# Autodesk Inventor assembly: chain(a)
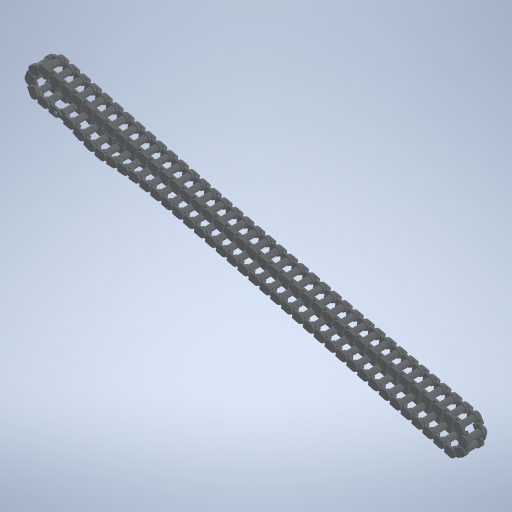
[picture p0: Inventor's stored thumbnail of the model, 512x512]
Saved by Autodesk Inventor 2023 (Build 270158000, 158)
## iProperties
Created: 2022-08-08
Part Number: chain(a)
Document SubType Name: Assembly
Designer: aaron
Author: aaron
## Documents named in this file (3)
- C:\Users\aaron\Documents\Inventor\Spin Up\library\Motion\New Sprockets\chain(a2).iam
- C:\Users\aaron\Documents\Inventor\Spin Up\library\Motion\New Sprockets\IQ chain.ipt
- C:\Users\aaron\Documents\Inventor\Spin Up\library\Motion\New Sprockets\8T.ipt
## Components (84 placed, 2 different names)
1. IQ chain:1 — Mate:2, Flush:3, Mate:64, Flush:65
2. IQ chain:2 — Mate:2, Flush:3, Mate:4, Flush:5
3. IQ chain:3 — Mate:4, Flush:5
4. IQ chain:4 — Mate:8, Flush:9
5. IQ chain:5 — Mate:8, Flush:9
6. IQ chain:6
7. IQ chain:7
8. IQ chain:8 — Mate:16, Flush:17
9. IQ chain:9 — Mate:16, Flush:17
10. IQ chain:10
11. IQ chain:11
12. IQ chain:12
13. IQ chain:13
14. IQ chain:14
15. IQ chain:15
16. IQ chain:16 — Mate:32, Flush:33
17. IQ chain:17 — Mate:32, Flush:33
18. IQ chain:18
19. IQ chain:19
20. IQ chain:20
21. IQ chain:21
22. IQ chain:22
23. IQ chain:23
24. IQ chain:24
25. IQ chain:25 — Mate:113, Flush:94
26. IQ chain:27 — Mate:113
27. IQ chain:28 — Flush:94
28. IQ chain:29 — Mate:120, Mate:125
29. IQ chain:33 — Mate:100, Flush:84
30. IQ chain:34
31. IQ chain:35
32. IQ chain:36
33. IQ chain:37
34. IQ chain:38
35. IQ chain:39
36. IQ chain:40
37. IQ chain:41
38. IQ chain:42
39. IQ chain:43
40. IQ chain:44
41. IQ chain:45
42. IQ chain:46
43. IQ chain:47
44. IQ chain:48
45. IQ chain:49
46. IQ chain:50
47. IQ chain:51 — Mate:118
48. IQ chain:52 — Mate:115
49. IQ chain:53 — Mate:116
50. IQ chain:54 — Mate:117
51. IQ chain:55
52. IQ chain:56
53. IQ chain:57
54. IQ chain:58
55. IQ chain:59
56. IQ chain:60
57. IQ chain:61
58. IQ chain:62
59. IQ chain:63
60. IQ chain:64 — Mate:64, Flush:65
61. IQ chain:70 — Mate:124, Mate:125
62. IQ chain:71 — Mate:122
63. IQ chain:72 — Mate:123
64. IQ chain:73 — Flush:95, Tangent:1
65. IQ chain:75 — Flush:95, Tangent:1
66. IQ chain:76 — Mate:109, Flush:93
67. IQ chain:77 — Mate:108, Flush:92
68. IQ chain:78
69. IQ chain:79
70. IQ chain:80
71. IQ chain:81
72. IQ chain:82
73. IQ chain:83 — Mate:100, Flush:84
74. IQ chain:84 — Mate:108, Flush:92
75. IQ chain:85 — Mate:110
76. IQ chain:86
77. IQ chain:87
78. IQ chain:88
79. IQ chain:89
80. IQ chain:90
81. IQ chain:91
82. IQ chain:92 — Mate:109, Flush:93, Mate:110
83. 8T:1 — Mate:114, Mate:115, Mate:116, Mate:117, Mate:118
84. 8T:2 — Mate:114, Mate:120, Mate:122, Mate:123, Mate:124
## Relationships (171: Mate 90, Flush 80, Tangent 1)
- Mate:2: IQ chain:1 ↔ IQ chain:2
- Flush:3: IQ chain:1 ↔ IQ chain:2
- [Mate]: IQ chain:3 ↔ IQ chain:4
- [Flush]: IQ chain:3 ↔ IQ chain:4
- Mate:4: IQ chain:2 ↔ IQ chain:3
- Flush:5: IQ chain:2 ↔ IQ chain:3
- [Mate]: IQ chain:5 ↔ IQ chain:6
- [Flush]: IQ chain:5 ↔ IQ chain:6
- [Mate]: IQ chain:7 ↔ IQ chain:8
- [Flush]: IQ chain:7 ↔ IQ chain:8
- [Mate]: IQ chain:6 ↔ IQ chain:7
- [Flush]: IQ chain:6 ↔ IQ chain:7
- Mate:8: IQ chain:4 ↔ IQ chain:5
- Flush:9: IQ chain:4 ↔ IQ chain:5
- [Mate]: IQ chain:9 ↔ IQ chain:10
- [Flush]: IQ chain:9 ↔ IQ chain:10
- [Mate]: IQ chain:11 ↔ IQ chain:12
- [Flush]: IQ chain:11 ↔ IQ chain:12
- [Mate]: IQ chain:10 ↔ IQ chain:11
- [Flush]: IQ chain:10 ↔ IQ chain:11
- [Mate]: IQ chain:13 ↔ IQ chain:14
- [Flush]: IQ chain:13 ↔ IQ chain:14
- [Mate]: IQ chain:15 ↔ IQ chain:16
- [Flush]: IQ chain:15 ↔ IQ chain:16
- [Mate]: IQ chain:14 ↔ IQ chain:15
- [Flush]: IQ chain:14 ↔ IQ chain:15
- [Mate]: IQ chain:12 ↔ IQ chain:13
- [Flush]: IQ chain:12 ↔ IQ chain:13
- Mate:16: IQ chain:8 ↔ IQ chain:9
- Flush:17: IQ chain:8 ↔ IQ chain:9
- [Mate]: IQ chain:17 ↔ IQ chain:18
- [Flush]: IQ chain:17 ↔ IQ chain:18
- [Mate]: IQ chain:19 ↔ IQ chain:20
- [Flush]: IQ chain:19 ↔ IQ chain:20
- [Mate]: IQ chain:18 ↔ IQ chain:19
- [Flush]: IQ chain:18 ↔ IQ chain:19
- [Mate]: IQ chain:21 ↔ IQ chain:22
- [Flush]: IQ chain:21 ↔ IQ chain:22
- [Mate]: IQ chain:23 ↔ IQ chain:24
- [Flush]: IQ chain:23 ↔ IQ chain:24
- [Mate]: IQ chain:22 ↔ IQ chain:23
- [Flush]: IQ chain:22 ↔ IQ chain:23
- [Mate]: IQ chain:20 ↔ IQ chain:21
- [Flush]: IQ chain:20 ↔ IQ chain:21
- [Mate]: IQ chain:27 ↔ IQ chain:28
- [Flush]: IQ chain:27 ↔ IQ chain:28
- [Mate]: IQ chain:28 ↔ IQ chain:29
- [Flush]: IQ chain:28 ↔ IQ chain:29
- [Mate]: IQ chain:24 ↔ IQ chain:25
- [Flush]: IQ chain:24 ↔ IQ chain:25
- Mate:32: IQ chain:16 ↔ IQ chain:17
- Flush:33: IQ chain:16 ↔ IQ chain:17
- [Mate]: IQ chain:33 ↔ IQ chain:34
- [Flush]: IQ chain:33 ↔ IQ chain:34
- [Mate]: IQ chain:35 ↔ IQ chain:36
- [Flush]: IQ chain:35 ↔ IQ chain:36
- [Mate]: IQ chain:34 ↔ IQ chain:35
- [Flush]: IQ chain:34 ↔ IQ chain:35
- [Mate]: IQ chain:37 ↔ IQ chain:38
- [Flush]: IQ chain:37 ↔ IQ chain:38
- [Mate]: IQ chain:39 ↔ IQ chain:40
- [Flush]: IQ chain:39 ↔ IQ chain:40
- [Mate]: IQ chain:38 ↔ IQ chain:39
- [Flush]: IQ chain:38 ↔ IQ chain:39
- [Mate]: IQ chain:36 ↔ IQ chain:37
- [Flush]: IQ chain:36 ↔ IQ chain:37
- [Mate]: IQ chain:41 ↔ IQ chain:42
- [Flush]: IQ chain:41 ↔ IQ chain:42
- [Mate]: IQ chain:43 ↔ IQ chain:44
- [Flush]: IQ chain:43 ↔ IQ chain:44
- [Mate]: IQ chain:42 ↔ IQ chain:43
- [Flush]: IQ chain:42 ↔ IQ chain:43
- [Mate]: IQ chain:45 ↔ IQ chain:46
- [Flush]: IQ chain:45 ↔ IQ chain:46
- [Mate]: IQ chain:47 ↔ IQ chain:48
- [Flush]: IQ chain:47 ↔ IQ chain:48
- [Mate]: IQ chain:46 ↔ IQ chain:47
- [Flush]: IQ chain:46 ↔ IQ chain:47
- [Mate]: IQ chain:44 ↔ IQ chain:45
- [Flush]: IQ chain:44 ↔ IQ chain:45
- [Mate]: IQ chain:40 ↔ IQ chain:41
- [Flush]: IQ chain:40 ↔ IQ chain:41
- [Mate]: IQ chain:49 ↔ IQ chain:50
- [Flush]: IQ chain:49 ↔ IQ chain:50
- [Mate]: IQ chain:51 ↔ IQ chain:52
- [Flush]: IQ chain:51 ↔ IQ chain:52
- [Mate]: IQ chain:50 ↔ IQ chain:51
- [Flush]: IQ chain:50 ↔ IQ chain:51
- [Mate]: IQ chain:53 ↔ IQ chain:54
- [Flush]: IQ chain:53 ↔ IQ chain:54
- [Mate]: IQ chain:55 ↔ IQ chain:56
- [Flush]: IQ chain:55 ↔ IQ chain:56
- [Mate]: IQ chain:54 ↔ IQ chain:55
- [Flush]: IQ chain:54 ↔ IQ chain:55
- [Mate]: IQ chain:52 ↔ IQ chain:53
- [Flush]: IQ chain:52 ↔ IQ chain:53
- [Mate]: IQ chain:57 ↔ IQ chain:58
- [Flush]: IQ chain:57 ↔ IQ chain:58
- [Mate]: IQ chain:59 ↔ IQ chain:60
- [Flush]: IQ chain:59 ↔ IQ chain:60
- [Mate]: IQ chain:58 ↔ IQ chain:59
- [Flush]: IQ chain:58 ↔ IQ chain:59
- [Mate]: IQ chain:61 ↔ IQ chain:62
- [Flush]: IQ chain:61 ↔ IQ chain:62
- [Mate]: IQ chain:63 ↔ IQ chain:64
- [Flush]: IQ chain:63 ↔ IQ chain:64
- [Mate]: IQ chain:62 ↔ IQ chain:63
- [Flush]: IQ chain:62 ↔ IQ chain:63
- [Mate]: IQ chain:60 ↔ IQ chain:61
- [Flush]: IQ chain:60 ↔ IQ chain:61
- [Mate]: IQ chain:56 ↔ IQ chain:57
- [Flush]: IQ chain:56 ↔ IQ chain:57
- [Mate]: IQ chain:48 ↔ IQ chain:49
- [Flush]: IQ chain:48 ↔ IQ chain:49
- Mate:64: IQ chain:1 ↔ IQ chain:64
- Flush:65: IQ chain:1 ↔ IQ chain:64
- [Mate]: IQ chain:70 ↔ IQ chain:71
- [Flush]: IQ chain:70 ↔ IQ chain:71
- [Mate]: IQ chain:72 ↔ IQ chain:73
- [Flush]: IQ chain:72 ↔ IQ chain:73
- [Mate]: IQ chain:71 ↔ IQ chain:72
- [Flush]: IQ chain:71 ↔ IQ chain:72
- [Mate]: IQ chain:75 ↔ IQ chain:76
- [Flush]: IQ chain:75 ↔ IQ chain:76
- [Mate]: IQ chain:77 ↔ IQ chain:78
- [Flush]: IQ chain:77 ↔ IQ chain:78
- [Mate]: IQ chain:79 ↔ IQ chain:80
- [Flush]: IQ chain:79 ↔ IQ chain:80
- [Mate]: IQ chain:78 ↔ IQ chain:79
- [Flush]: IQ chain:78 ↔ IQ chain:79
- [Mate]: IQ chain:81 ↔ IQ chain:82
- [Flush]: IQ chain:81 ↔ IQ chain:82
- [Mate]: IQ chain:82 ↔ IQ chain:83
- [Flush]: IQ chain:82 ↔ IQ chain:83
- [Mate]: IQ chain:80 ↔ IQ chain:81
- [Flush]: IQ chain:80 ↔ IQ chain:81
- Mate:100: IQ chain:33 ↔ IQ chain:83
- Flush:84: IQ chain:33 ↔ IQ chain:83
- [Mate]: IQ chain:85 ↔ IQ chain:86
- [Flush]: IQ chain:85 ↔ IQ chain:86
- [Mate]: IQ chain:87 ↔ IQ chain:88
- [Flush]: IQ chain:87 ↔ IQ chain:88
- [Mate]: IQ chain:86 ↔ IQ chain:87
- [Flush]: IQ chain:86 ↔ IQ chain:87
- [Mate]: IQ chain:89 ↔ IQ chain:90
- [Flush]: IQ chain:89 ↔ IQ chain:90
- [Mate]: IQ chain:90 ↔ IQ chain:91
- [Flush]: IQ chain:90 ↔ IQ chain:91
- [Mate]: IQ chain:88 ↔ IQ chain:89
- [Flush]: IQ chain:88 ↔ IQ chain:89
- [Mate]: IQ chain:84 ↔ IQ chain:91
- [Flush]: IQ chain:84 ↔ IQ chain:91
- Mate:108: IQ chain:77 ↔ IQ chain:84
- Flush:92: IQ chain:77 ↔ IQ chain:84
- Mate:109: IQ chain:76 ↔ IQ chain:92
- Flush:93: IQ chain:76 ↔ IQ chain:92
- Mate:110: IQ chain:85 ↔ IQ chain:92
- Mate:113: IQ chain:25 ↔ IQ chain:27
- Mate:114 (235.712 mm): 8T:1 ↔ 8T:2
- Mate:115: IQ chain:52 ↔ 8T:1
- Mate:116: IQ chain:53 ↔ 8T:1
- Mate:117: IQ chain:54 ↔ 8T:1
- Mate:118: IQ chain:51 ↔ 8T:1
- Flush:94: IQ chain:25 ↔ IQ chain:28
- Mate:120: IQ chain:29 ↔ 8T:2
- Mate:122: IQ chain:71 ↔ 8T:2
- Mate:123: IQ chain:72 ↔ 8T:2
- Mate:124: IQ chain:70 ↔ 8T:2
- Mate:125: IQ chain:29 ↔ IQ chain:70
- Flush:95: IQ chain:73 ↔ IQ chain:75
- Tangent:1: IQ chain:73 ↔ IQ chain:75
## Named parameters: d5_d3 = 0 mm, d6_d4 = 0 mm, d9_d3 = 0 mm, d10_d4 = 0 mm, d11_d5_d3 = 0 mm, d12_d6_d4 = 0 mm, d13_d7 = 0 mm, d14_d8 = 0 mm, d17_d3 = 0 mm, d18_d4 = 0 mm, d19_d5_d3 = 0 mm, d20_d6_d4 = 0 mm, d21_d7 = 0 mm, d22_d8 = 0 mm, d23_d9_d3 = 0 mm, d24_d10_d4 = 0 mm, d25_d11_d5_d3 = 0 mm, d26_d12_d6_d4 = 0 mm, d27_d13_d7 = 0 mm, d28_d14_d8 = 0 mm, d29_d15 = 0 mm, d30_d16 = 0 mm, d33_d32 = 0 mm, d34_d3 = 0 mm, d35_d4 = 0 mm, d36_d5_d3 = 0 mm, d37_d6_d4 = 0 mm, d38_d7 = 0 mm, d39_d8 = 0 mm, d40_d9_d3 = 0 mm, d41_d10_d4 = 0 mm, d42_d11_d5_d3 = 0 mm, d43_d12_d6_d4 = 0 mm, d44_d13_d7 = 0 mm, d45_d14_d8 = 0 mm, d46_d15 = 0 mm, d47_d16 = 0 mm, d50_d19_d5_d3 = 0 mm, d51_d20_d6_d4 = 0 mm, d60_d29_d15 = 0 mm, d61_d30_d16 = 0 mm, d62_d31 = 0 mm, d65_d32 = 0 mm, d66_d33_d32 = 0 mm, d67_d34_d3 = 0 mm, d68_d35_d4 = 0 mm, d69_d36_d5_d3 = 0 mm, d70_d37_d6_d4 = 0 mm, d71_d38_d7 = 0 mm, d72_d39_d8 = 0 mm, d73_d40_d9_d3 = 0 mm, d74_d41_d10_d4 = 0 mm, d75_d42_d11_d5_d3 = 0 mm, d76_d43_d12_d6_d4 = 0 mm, d77_d44_d13_d7 = 0 mm, d78_d45_d14_d8 = 0 mm, d79_d46_d15 = 0 mm, d80_d47_d16 = 0 mm, d81_d48_d17_d3 = 0 mm, d82_d49_d18_d4 = 0 mm, d83_d50_d19_d5_d3 = 0 mm, d84_d51_d20_d6_d4 = 0 mm, d85_d52_d21_d7 = 0 mm, d86_d53_d22_d8 = 0 mm, d87_d54_d23_d9_d3 = 0 mm, d88_d55_d24_d10_d4 = 0 mm, d89_d56_d25_d11_d5_d3 = 0 mm, d90_d57_d26_d12_d6_d4 = 0 mm, d91_d58_d27_d13_d7 = 0 mm, d92_d59_d28_d14_d8 = 0 mm, d93_d60_d29_d15 = 0 mm, d94_d61_d30_d16 = 0 mm, d95_d62_d31 = 0 mm, d96_d63 = 0 mm, d97_d64 = 0 mm, d98_d3 = 0 mm, d99_d4 = 0 mm, d100_d5_d3 = 0 mm, d101_d6_d4 = 0 mm, d102_d7 = 0 mm, d103_d8 = 0 mm, d104_d9_d3 = 0 mm, d105_d10_d4 = 0 mm, d106_d11_d5_d3 = 0 mm, d107_d12_d6_d4 = 0 mm, d108_d13_d7 = 0 mm, d109_d14_d8 = 0 mm, d110_d15 = 0 mm, d111_d16 = 0 mm, d112_d17_d3 = 0 mm, d113_d18_d4 = 0 mm, d114_d19_d5_d3 = 0 mm, d115_d20_d6_d4 = 0 mm, d116_d21_d7 = 0 mm, d117_d22_d8 = 0 mm, d118_d23_d9_d3 = 0 mm, d119_d24_d10_d4 = 0 mm, d120_d25_d11_d5_d3 = 0 mm, d121_d26_d12_d6_d4 = 0 mm, d122_d27_d13_d7 = 0 mm, d123_d28_d14_d8 = 0 mm, d124_d29_d15 = 0 mm, d125_d30_d16 = 0 mm, d126_d31 = 0 mm, d136_d38_d7 = 0 mm, d137_d39_d8 = 0 mm, d146_d23_d9_d3 = 0 mm, d147_d24_d10_d4 = 0 mm, d148_d25_d11_d5_d3 = 0 mm, d149_d26_d12_d6_d4 = 0 mm, d150_d27_d13_d7 = 0 mm, d151_d28_d14_d8 = 0 mm, d170_d98_d3 = 0 mm, d171_d99_d4 = 0 mm, d172_d100_d5_d3 = 0 mm, d173_d101_d6_d4 = 0 mm, d174_d102_d7 = 0 mm, d175_d103_d8 = 0 mm, d176_d104_d9_d3 = 0 mm, d177_d105_d10_d4 = 0 mm, d178_d108_d13_d7 = 0 mm, d179_d109_d14_d8 = 0 mm, d180_d110_d15 = 0 mm, d181_d111_d16 = 0 mm, d184_d170_d98_d3 = 0 mm, d185_d171_d99_d4 = 0 mm, d186_d172_d100_d5_d3 = 0 mm, d187_d173_d101_d6_d4 = 0 mm, d188_d174_d102_d7 = 0 mm, d189_d175_d103_d8 = 0 mm, d190_d176_d104_d9_d3 = 0 mm, d191_d177_d105_d10_d4 = 0 mm, d192_d178_d108_d13_d7 = 0 mm, d193_d179_d109_d14_d8 = 0 mm, d194_d180_d110_d15 = 0 mm, d195_d181_d111_d16 = 0 mm, d196_d182 = 0 mm, d197_d183 = 0 mm
